# Autodesk Inventor assembly: 0.75DXPSRS04.00S100_0010000000S100_001 000000
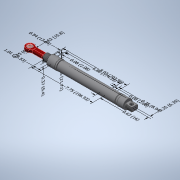
[picture p0: Inventor's stored thumbnail of the model, 180x180]
Saved by Autodesk Inventor 2022.3 (Build 263350000, 350)
## iProperties
Category: PARTsolutions
Company: PARKERHANNIFIN
Created: 2023-02-15
Part Number: 0.75DXPSRS04.00S100_0010000000S100_001 000000
Catalog Web Link: www.cadenas.de
Description: SR Series-Pneumatic Cylinder
Vendor: PARKERHANNIFIN
Document SubType Name: Assembly
Designer: psAdmin
Manufacturer: PARKERHANNIFIN
Mass: 46.0414 g
Surface Area: 325.33 cm^2
Volume: 39.8302 cm^3
Density: 1.15594 g/cm^3
PSOL_IDENT_0: {$CADENAS_DATA/23d-libs/parkerpdn/actuators_cylinders/pneumatic_cylinders/sr_series/sr_asmtab.prj},4
PSOL_IDENT_1: 42 {VTYP=3D},{STYP=ASSTAB},{NB=0.75DXPSRS04.00S100_0010000000S100_001 000000},{LINA=0.75DXPSRS04.00}
PSOL_IDENT_2: ,{NN=SR Series},{DATE=24.02.2022 20:39:50},{GEOMDATE=02.09.2021 11:25:18},{VERSION=},{LINEID=10},{WB
PSOL_IDENT_3: VAR=BORE,CUH,DR,MNT,SERIES,PISTON,SEALS,RODMAT,RES,RETS,RETT,RET,READ,REEL,RWF,RESE2,RETE2,RETTE2,RE
PSOL_IDENT_4: TSE2,REAE2,REELE2,RWFE2,CUC,STROKE,SPEC,PLH,PLC,NLH,NLC,LENGTH,MCD,RS,RRPT,RRPH,ARB,ORPP},{WBNUMERIC=
PSOL_IDENT_5: BORE,READ,REEL,REAE2,REELE2,STROKE,LENGTH}  {NB=0.75DXPSRS04.00S100_0010000000S100_001 000000},{LINA=
PSOL_IDENT_6: 0.75DXPSRS04.00},{KT=DUMMY},{PN=0.75DXPSRS04.00},{PR=SR Series},{BORE=0.75},{BOREPN=0.75},{BOREPN1=0
PSOL_IDENT_7: .75},{BORECON1=0.7500},{CUH=_},{CUHALG='_' , 'No Cushion Head' , 'C' , 'C - Cushion Head' },{CUHCON=
PSOL_IDENT_8: },{DR=_},{DRALG= <'_' , 'Single Rod'> , 'K' , 'K - Double Rod' },{DRCON=},{MNT=DXP},{MNTALG= 'N' , '
PSOL_IDENT_9: N - Nose Mount, Spring Return' , 'NR' , 'NR - Nose Mount, Spring Return, Hex Rod (non-rotating)' , '
PSOL_IDENT_10: NRP' , 'NRP - Pivot and Nose Mount, Spring Return, Hex Rod (non-rotating)' , 'P' , 'P - Pivot Mount,
PSOL_IDENT_11: Spring Return' , 'R' , 'R - Nose Mount, Spring Extended' , 'RP' , 'RP - Pivot and Nose Mount, Sprin
PSOL_IDENT_12: g Extend' , 'D' , 'D - Nose Mount, Double Acting'  , 'DP' , 'DP - Pivot and Nose Mount, Double Actin
PSOL_IDENT_13: g, Pivot Pin' , 'DXP' , 'DXP - Pivot and Nose Mount, Double Acting, No Pivot Pin' ,  'A' , 'A - Nose
PSOL_IDENT_14: Mount, Spring Return, Head Adjustable Stroke' , 'RA' , 'RA - Nose Mount, Spring Extend, Cap Adjusta
PSOL_IDENT_15: ble Stroke' , 'AP' , 'AP - Pivot Mount, Spring Return, Head Adjustable Stroke' , 'AR' , 'AR - Air Re
PSOL_IDENT_16: servoirs' , 'BRN' , 'BRN - Rear Block Mount, Single Acting, Spring Return' , 'BRR' , 'BRR - Rear Blo
PSOL_IDENT_17: ck Mount, Single Acting, Spring Extend' , 'BFD' , 'BFD - Front Block Mount, Double Acting' , 'BRD' ,
PSOL_IDENT_18: 'BRD - Rear Block Mount, Double Acting' , 'BFN' , 'BFN - Front Block Mount, Single Acting, Spring R
PSOL_IDENT_19: eturn' , 'BFR' , 'BFR - Front Block Mount, Single Acting, Spring Extend' , 'TRN' , 'TRN - Rear Trunn
PSOL_IDENT_20: ion Mount, Single Acting, Spring Return' , 'TRR' , 'TRR - Rear Trunnion Mount, Single Acting, Spring
PSOL_IDENT_21: Extend' , 'TFD' , 'TFD - Front Trunnion Mount, Double Acting' , 'TRD' , 'TRD - Rear Trunnion Mount,
PSOL_IDENT_22: Double Acting' , 'TFN' , 'TFN - Front Trunnion Mount, Single Acting, Spring Return' , 'TFR' , 'TFR
PSOL_IDENT_23: - Front Trunnion Mount, Single Acting, Spring Extend' },{CT=Double acting},{SERIES=SR},{SERIESALG= '
PSOL_IDENT_24: SR' , 'SR - Non-Repairable Cylinder'  ,'SRM','SRM - Non-Repairable Cylinder with Magnet'  ,'SRD','SR
PSOL_IDENT_25: D - Non-Repairable Cylinder with Delrin Caps'  ,'SRDM','SRDM - Non-Repairable Cylinder with Delrin C
PSOL_IDENT_26: aps and Magnet'  , 'SRG' , 'SRG - Non-Repairable Cylinder with Stainless Steel Caps'  , 'SRGM' , 'SR
PSOL_IDENT_27: GM - Non-Repairable Cylinder with Stainless Steel Caps and Magnet' },{SERIESCON=SR},{SVAL1= 'SR' , '
PSOL_IDENT_28: SR - Non-Repairable Cylinder' },{SVAL2= ,'SRM','SRM - Non-Repairable Cylinder with Magnet' },{SVAL3=
PSOL_IDENT_29: ,'SRD','SRD - Non-Repairable Cylinder with Delrin Caps' },{SVAL4= ,'SRDM','SRDM - Non-Repairable Cy
PSOL_IDENT_30: linder with Delrin Caps and Magnet' },{SVAL5= , 'SRG' , 'SRG - Non-Repairable Cylinder with Stainles
PSOL_IDENT_31: s Steel Caps' },{SVAL6= , 'SRGM' , 'SRGM - Non-Repairable Cylinder with Stainless Steel Caps and Mag
PSOL_IDENT_32: net' },{PISTON=_},{PISTONALG= <'_' , 'No Bumpers'> , 'B' , 'B - With Bumpers' },{PISTONALGOLD= <'_'
PSOL_IDENT_33: , 'No Bumpers'> , 'B' , 'B - With Bumpers' },{PISTONDESC=0},{PISTONPN=},{PISTONCON=},{SEALS=_},{SEAL
PSOL_IDENT_34: SALG= <'_' , 'Standard Seals'> , 'V' , 'V - Flourocarbon Seals'  ,'W' , 'W - Rod Wiper'  },{SEALSCON=
PSOL_IDENT_35: },{RWOPT= ,'W' , 'W - Rod Wiper' },{SPECIAL=},{RODMAT=},{RODMATALG= '' , 'Stainless Steel' },{RODMAT
PSOL_IDENT_36: CON=},{RES=_},{RETS=},{RETALG='','N/A'},{RETT=},{RETTALG='','N/A'},{RET=},{RETSALG='','N/A'},{READ=0
PSOL_IDENT_37: },{REAMAX=2.5},{REAALG=[0]},{REE=N/A},{REEMIN=0.440},{REEL=0.000},{REELALG=[0]},{RWF=},{RWFALG='','N
PSOL_IDENT_38: /A'},{RETE2ALG='','N/A'},{PREE2ALG= '_' , 'N/A' },{RESE2=_},{RETE2=},{RETTE2=},{RETTE2ALG='','N/A'},
PSOL_IDENT_39: {RETSE2=},{RETSE2ALG='','N/A'},{REAE2=0},{REAE2ALG=[0]},{REEE2=N/A},{REELE2=0.000},{REELE2ALG=[0]},{
PSOL_IDENT_40: RWFE2=},{RWFE2ALG='','N/A'},{PREALG= <'_' , 'Standard Piston Rod End'> , '3' , '3 - Non-Standard Pis
PSOL_IDENT_41: ton Rod End' },{PRECON=},{CUC=_},{CUCALG= <'_' , 'No Cushion Cap'> , 'C' , 'C - Cushion Cap' },{CUCC
PSOL_IDENT_42: ON=},{STROKE=4.00},{STROKEALG=[0.1:34/0.01]},{SPEC=S},{STROKEMIN=0.1},{STROKEMAX=34},{PLH=1},{PLC=1}
PSOL_IDENT_43: ,{NLH=},{NLC=},{LENGTH=0.00},{LENALG=0},{LENMIN=0.12},{LENMAX=2},{A=0.50},{A1=0.5},{AA=0.86},{AA1=0.
PSOL_IDENT_44: 81},{AA2=0.86},{AF=0.00},{AF1=0},{AS=0.00},{AS1=-0.03},{B=0.622},{BC=0.00},{C=0.00},{C1=0.25},{CC=0.
PSOL_IDENT_45: 25},{CF=0.00},{CP=0.00},{CS=0.00},{CS1=1.69},{D=0.00},{D1=0.22},{D2=0.25},{DA=-},{DB=0.00},{E=0.37},
PSOL_IDENT_46: {E1=0.37},{E2=1},{EE=1/8 NPTF},{EE1=1/8 NPTF},{F=0.00},{F1=0.47},{FH=0.00},{GH=0.00},{GM=0.00},{GW=0
PSOL_IDENT_47: .00},{HP=0.00},{J=0.19},{J1=0.19},{KK=1/4-28 UNF},{KM=5/8-18},{KM1=1/2-20},{KM2=5/8-18},{KP=-},{KP1=
PSOL_IDENT_48: 5/8-18 UNF},{L=0.34},{L1=0.34},{MB=0.00},{MB1=1.12},{MT=0.00},{NM=0.00},{PP=0.62},{PP1=0.62},{Q=0.00
PSOL_IDENT_49: },{Q1=0.81},{R=0.00},{R1=0},{RM=0.00},{RW=0.00},{TM=0.00},{S=-},{S1=#10-32 UNC},{SB=0},{SC=-},{SE=0.
PSOL_IDENT_50: 00},{SE1=0.44},{SE2=0.5},{SO=-},{SW=0.00},{T=0.00},{T1=0.62},{TD=0.000},{TD1=0.25},{TL=0.00},{UT=0.0
PSOL_IDENT_51: 0},{UT1=0.75},{V=0.08},{W=0.50},{W1=0.69},{W2=0.5},{WH=0.00},{WH1=0.97},{WH2=0.97},{Y=0.97},{Y1=0},{
PSOL_IDENT_52: Y2=0.97},{X=0.00},{X1=1.69},{X2=2.69},{TT=0.00},{TTDX1=4},{TTDX2=4},{XJ=3.75},{XJNRP1=2.53},{XJNRP2=
PSOL_IDENT_53: 2.78},{XJP1=2.28},{XJP2=2.53},{XJRP1=2.44},{XJRP2=2.69},{XJDP1=3.75},{XJDP2=3.75},{XJDXP1=3.75},{XJD
PSOL_IDENT_54: XP2=3.75},{XJAP1=3.6},{XJTRN1=1.94},{XJTRN2=2.19},{XJTRR1=2.85},{XJTRR2=3.1},{XJTFD1=0.69},{XJTRD1=3
PSOL_IDENT_55: .41},{XJTRD2=3.41},{XJTFN1=0.69},{XJTFR1=0.69},{Z=0.252},{Z1=0.252},{ZJ=4.03},{ZJN1=1.5},{ZJN2=1.75}
PSOL_IDENT_56: ,{ZJNR1=1.75},{ZJNR2=2},{ZJNRP1=2.81},{ZJNRP2=3.06},{ZJP1=2.56},{ZJP2=2.81},{ZJR1=2.31},{ZJR2=2.56},
PSOL_IDENT_57: {ZJRP1=2.72},{ZJRP2=2.97},{ZJD1=2.97},{ZJD2=2.97},{ZJDP1=4.03},{ZJDP2=4.03},{ZJDXP1=4.03},{ZJDXP2=4.
PSOL_IDENT_58: 03},{ZJDX1=4.03},{ZJA1=3.12},{ZJRA1=2.242},{ZJAP1=3.88},{ZJBRN1=2.31},{ZJBRN2=2.56},{ZJBRR1=3.22},{Z
PSOL_IDENT_59: JBRR2=3.47},{ZJBFD1=3.22},{ZJBFD2=3.22},{ZJBRD1=3.78},{ZJBRD2=3.78},{ZJBFN1=2.66},{ZJBFN2=2.91},{ZJB
PSOL_IDENT_60: FR1=2.56},{ZJBFR2=2.81},{ZJAR=1.938},{ADDER=0.000},{SRSR=0.125},{SESR=0.125},{DASR=0},{KSR=0},{SRSRM=
PSOL_IDENT_61: 0.125},{SESRM=0.125},{DASRM=0.25},{KSRM=0.312},{ASR=3.4},{ASRM=3.4},{PPATH=parts/sr_asmtpl.prj},{TEX
PSOL_IDENT_62: T2D=0.075},{SPACE2D=0.075},{STRLENPN=04.00},{STRLENPN1=4.00},{STRLENPN2=.00},{PRA=DXP},{STRK2D=0.000
PSOL_IDENT_63: },{X2D=1.5},{STROKESW=4},{LENGTHSW=0},{X2DD=0},{CUSHIONHEAD=No},{CUSHIONCAP=No},{RODTYPE=SR},{CYLTYP
PSOL_IDENT_64: E=DA},{PISTONTYPE=NP},{DXFLIB=da_sr.dxf},{BUSH=SR},{STROKEPN=4.00},{STROKEPN1=04},{PLHALG='1','Port
PSOL_IDENT_65: Position 1 Head End','2','Port Position 2 Head End','3','Port Position 3 Head End','4','Port Positio
PSOL_IDENT_66: n 4 Head End'},{PLCALG='1','Port Position 1 Cap End','2','Port Position 2 Cap End','3','Port Positio
PSOL_IDENT_67: n 3 Cap End','4','Port Position 4 Cap End'},{NLHALG='','N/A'},{NLCALG='','N/A'},{RODLEN=8.03},{REEE2
PSOL_IDENT_68: MIN=0.440},{PNS=0.75DXPSRS04.00S100_0010000000},{MCDALG= '0','No','1','Yes' },{MCD=0},{RSALG= '0','N
PSOL_IDENT_69: o','1','Yes' },{RS=0},{RRPT=0},{RRPTALG='0','No','1','Remove rear pivot tang.'},{RRPHALG='0','No','1'
PSOL_IDENT_70: ,'Ream pivot pin hole'},{RRPH=0},{ARBALG='0','No','1','Add pivot bushing (standard dia.)'},{ARB=0},{
PSOL_IDENT_71: OPPALG='0','No','1','Omit rear pivot pin.'},{P1=1},{ORPP=0},{SPECPN=S}
NB: 0.75DXPSRS04.00S100_0010000000S100_001 000000
NN: SR Series
NT: Pneumatic Cylinder
NBSYN: $PNS.$SPEC.$PLH.$RETS.$RETT.$RET.$READ.$REEL.$RWF.$RESE2.$RETE2.$RETTE2.$RETSE2.$REAE2.$REELE2.$RWFE2.$PLC.$NLH.$NLC. $RS.$MCD.$RRPT.$RRPH.$ARB.$ORPP.
LINA: 0.75DXPSRS04.00
CATALOG: Parker Pneumatic Division
PN: 0.75DXPSRS04.00
PR: SR Series
BORE: 0.75
CUH: No Cushion Head
DR: Single Rod
MNT: DXP - Pivot and Nose Mount, Double Acting, No Pivot Pin
SERIES: SR - Non-Repairable Cylinder
PISTON: No Bumpers
SEALS: Standard Seals
RODMAT: Stainless Steel
RES: Standard Piston Rod End
RETS: N/A
RETT: N/A
RET: N/A
READ: 0
REE: N/A
REEL: 0
RWF: N/A
RESE2: N/A
RETE2: N/A
RETTE2: N/A
RETSE2: N/A
REAE2: 0
REEE2: N/A
REELE2: 0
RWFE2: N/A
CUC: No Cushion Cap
STROKE: 4
SPEC: Special Modifications
PLH: Port Position 1 Head End
PLC: Port Position 1 Cap End
NLH: N/A
NLC: N/A
LENGTH: 0
A: 0.5
AA: 0.86
AF: 0
AS: 0
B: 0.622
BC: 0
C: 0
CC: 0.25
CF: 0
CP: 0
CS: 0
D: 0
DA: -
DB: 0
E: 0.37
EE: 1/8 NPTF
F: 0
FH: 0
GH: 0
GM: 0
GW: 0
HP: 0
J: 0.19
KK: 1/4-28 UNF
KM: 5/8-18
KP: -
L: 0.34
MB: 0
MT: 0
NM: 0
PP: 0.62
Q: 0
R: 0
RM: 0
RW: 0
TM: 0
S: -
SB: 0
SC: -
SE: 0
SO: -
SW: 0
T: 0
TD: 0
TL: 0
UT: 0
V: 0.08
W: 0.5
WH: 0
Y: 0.97
X: 0
TT: 0
XJ: 3.75
Z: 0.252
ZJ: 4.03
STRK2D: 0
MCD: No
RS: No
RRPT: No
RRPH: No
ARB: No
ORPP: No
SUPPLIER: PARKERHANNIFIN
ARTICLENO: 0.75DXPSRS04.00S100_0010000000S100_001 000000
BOMINFO: 0.75DXPSRS04.00
CREATOR: CADENAS GmbH
Title: 0.75DXPSRS04.00
Author: Cadenas PARTsolutions
Comments: Pneumatic Cylinder
## Documents named in this file (7)
- C:\Users\23kaltomare\Desktop\2023-Charged-Up\COMMON PARTS\AIR CYLINDERS\Parker\3_4_Bore_4_Stroke_PARKERPDN_075DXPSRS0400S\AIS2022\0_75DXPSRS04_00S100_0010000000S100_001 000000.iam
- C:\Users\23kaltomare\Desktop\2023-Charged-Up\COMMON PARTS\AIR CYLINDERS\Parker\3_4_Bore_4_Stroke_PARKERPDN_075DXPSRS0400S\AIS2022\0_75DXPSR4HLEN1_38CLEN1_347HOLEN1_595COLEN1_562N0000SR_dummy11SAM00_00.ipt
- C:\Users\23kaltomare\Desktop\2023-Charged-Up\COMMON PARTS\AIR CYLINDERS\Parker\3_4_Bore_4_Stroke_PARKERPDN_075DXPSRS0400S\AIS2022\0_75DXP-H_SRS1.ipt
- C:\Users\23kaltomare\Desktop\2023-Charged-Up\COMMON PARTS\AIR CYLINDERS\Parker\3_4_Bore_4_Stroke_PARKERPDN_075DXPSRS0400S\AIS2022\0_75-5_303x0_810_body.ipt
- C:\Users\23kaltomare\Desktop\2023-Charged-Up\COMMON PARTS\AIR CYLINDERS\Parker\3_4_Bore_4_Stroke_PARKERPDN_075DXPSRS0400S\AIS2022\0_75DXP-C_SRS10.ipt
- C:\Users\23kaltomare\Desktop\2023-Charged-Up\COMMON PARTS\AIR CYLINDERS\Parker\3_4_Bore_4_Stroke_PARKERPDN_075DXPSRS0400S\AIS2022\6_4680_8730_50_500Double acting_00_006_4680_500_75N.ipt
- C:\Users\23kaltomare\Desktop\2023-Charged-Up\COMMON PARTS\AIR CYLINDERS\TieRod End\60685K321_PTFE-LINED ALUMINUM BALL JOINT ROD END.ipt
## Components (6 placed, 6 different names)
1. 0_75DXPSR4HLEN1_38CLEN1_347HOLEN1_595COLEN1_562N0000SR_dummy11SAM00_00:1
2. 0_75DXP-H_SRS1:1 — Insert:1
3. 0_75-5_303x0_810_body:1
4. 0_75DXP-C_SRS10:1 — Angle:1
5. 6_4680_8730_50_500Double acting_00_006_4680_500_75N:1 — Insert:1, Insert:2
6. 60685K321_PTFE-LINED ALUMINUM BALL JOINT ROD END:1 — Insert:2, Angle:1
## Relationships (3: Insert 2, Angle 1)
- Insert:1: 0_75DXP-H_SRS1:1 ↔ 6_4680_8730_50_500Double acting_00_006_4680_500_75N:1
- Insert:2 (-9.525 mm): 6_4680_8730_50_500Double acting_00_006_4680_500_75N:1 ↔ 60685K321_PTFE-LINED ALUMINUM BALL JOINT ROD END:1
- Angle:1 (0 deg): 0_75DXP-C_SRS10:1 ↔ 60685K321_PTFE-LINED ALUMINUM BALL JOINT ROD END:1
